# Autodesk Inventor assembly: stay11
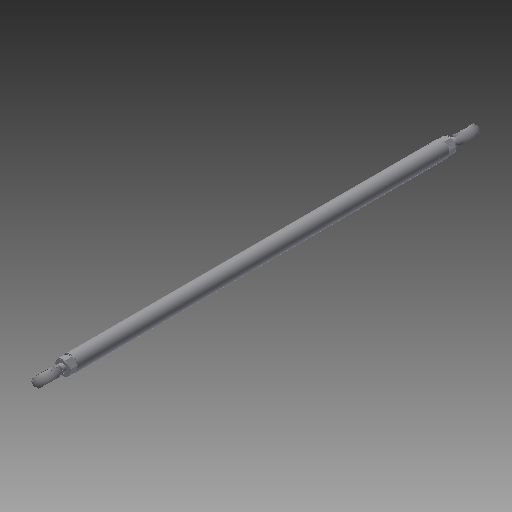
[picture p0: Inventor's stored thumbnail of the model, 512x512]
Saved by Autodesk Inventor 2018.2 (Build 222227000, 227)
## iProperties
Created: 2018-04-27
Part Number: stay11
Material: 一般
Document SubType Name: Assembly
Designer: ku_sk
Author: ku_sk
## Documents named in this file (3)
- C:\Users\ku_sk\Documents\Inventor\Aero\KS-15\Rr.wing\parts\stay\stay11.iam
- C:\Users\ku_sk\Documents\Inventor\Aero\KS-15\Rr.wing\parts\stay\pipe_16mm_360mm1.ipt
- C:\Users\ku_sk\Documents\Inventor\Aero\KS-15\Rr.wing\parts\stay\end\stay end1.iam
## Components (3 placed, 2 different names)
1. pipe_16mm_360mm1:1 — メイト:3, メイト:2, メイト:1, メイト:5, メイト:4, メイト:7, メイト:6
2. stay end1:1 [sub-assembly] — メイト:5, メイト:4
3. stay end1:2 [sub-assembly] — メイト:7, メイト:6
## Relationships (7: Mate 7)
- メイト:3 [Mate]: pipe_16mm_360mm1:1
- メイト:2 [Mate]: pipe_16mm_360mm1:1
- メイト:1 [Mate]: pipe_16mm_360mm1:1
- メイト:5 [Mate]: pipe_16mm_360mm1:1 ↔ stay end1:1
- メイト:4 [Mate]: pipe_16mm_360mm1:1 ↔ stay end1:1
- メイト:7 [Mate]: pipe_16mm_360mm1:1 ↔ stay end1:2
- メイト:6 [Mate]: pipe_16mm_360mm1:1 ↔ stay end1:2
